# Autodesk Inventor assembly: VersaRoller Generator V2
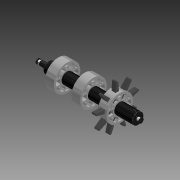
[picture p0: Inventor's stored thumbnail of the model, 180x180]
Saved by Autodesk Inventor 2022 (Build 260153000, 153)
## iProperties
Created: 2022-02-17
Part Number: VersaRoller Generator V2
Document SubType Name: Assembly
Designer: Desktop
Author: Desktop
## Documents named in this file (7)
- E:\Middleton Robotics\Collaborative Robots\Collaborative Part Library\Roller Systems\VersaRoller Generator V2.iam
- E:\Middleton Robotics\Collaborative Robots\Collaborative Part Library\Roller Systems\VersaTube Generator.ipt
- E:\Middleton Robotics\Collaborative Robots\Collaborative Part Library\Roller Systems\WCP Star Flex Wheel.ipt
- E:\Middleton Robotics\Collaborative Robots\Collaborative Part Library\Wheels\Compliant Wheel Generator\3 in 30A 1.125 in Hex Compliant Wheel VEX.ipt
- E:\Middleton Robotics\Collaborative Robots\Collaborative Part Library\Wheels\Compliant Wheel Generator.ipt
- E:\Middleton Robotics\Collaborative Robots\Collaborative Part Library\Roller Systems\VersaRoller End Cap.ipt
- E:\Middleton Robotics\Collaborative Robots\Collaborative Part Library\Roller Systems\VersaTube Generator\10 in Metal VersaRoller Driven No Surgical Tubing.ipt
## Components (7 placed, 4 different names)
1. 10 in Metal VersaRoller Driven No Surgical Tubing:1 — Mate:1, Flush:1, Flush:2, Flush:3, Insert:3, Mate:2, Insert:4, Mate:3
2. VersaRoller End Cap:1 — Insert:3, Mate:2
3. VersaRoller End Cap:2 — Insert:4, Mate:3
4. WCP Star Flex Wheel:1 — Insert:1
5. 3 in 30A 1.125 in Hex Compliant Wheel VEX:1 — Mate:1, Insert:1, Flush:4
6. 3 in 30A 1.125 in Hex Compliant Wheel VEX:2
7. 3 in 30A 1.125 in Hex Compliant Wheel VEX:3
## Component patterns: (3 elements, first: 3 in 30A 1.125 in Hex Compliant Wheel VEX:1)
## Relationships (10: Flush 4, Mate 3, Insert 3)
- Mate:1: 10 in Metal VersaRoller Driven No Surgical Tubing:1 ↔ 3 in 30A 1.125 in Hex Compliant Wheel VEX:1
- Insert:1 (6.35 mm): WCP Star Flex Wheel:1 ↔ 3 in 30A 1.125 in Hex Compliant Wheel VEX:1
- Flush:1: 10 in Metal VersaRoller Driven No Surgical Tubing:1
- Flush:2: 10 in Metal VersaRoller Driven No Surgical Tubing:1
- Flush:3: 10 in Metal VersaRoller Driven No Surgical Tubing:1
- Insert:3: 10 in Metal VersaRoller Driven No Surgical Tubing:1 ↔ VersaRoller End Cap:1
- Mate:2: 10 in Metal VersaRoller Driven No Surgical Tubing:1 ↔ VersaRoller End Cap:1
- Insert:4: 10 in Metal VersaRoller Driven No Surgical Tubing:1 ↔ VersaRoller End Cap:2
- Mate:3: 10 in Metal VersaRoller Driven No Surgical Tubing:1 ↔ VersaRoller End Cap:2
- Flush:4 (76.2 mm): 3 in 30A 1.125 in Hex Compliant Wheel VEX:1
## Named parameters: TubeLength = 254 mm, Wheels = 3, Remainder = 38.1 mm, Offset = 76.2 mm
